# Autodesk Inventor assembly: microven
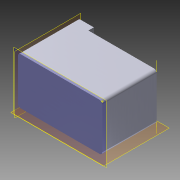
[picture p0: Inventor's stored thumbnail of the model, 180x180]
Saved by Autodesk Inventor 2015 (Build 190159000, 159)
## iProperties
Created: 2015-10-18
Part Number: microven
Document SubType Name: Assembly
Designer: omae
Author: omae
## Documents named in this file (2)
- C:\Users\omae\Desktop\研究室\論文・資料\ROS\kitchen\stl\microven.iam
- C:\Users\omae\Desktop\研究室\論文・資料\ROS\kitchen\toolinstall\homeIsland\summerSeminar\micorooven\microwaveOvenBox.ipt
## Components (1 placed, 1 different names)
1. microwaveOvenBox:1 — メイト:1, メイト:2, メイト:3
## Relationships (3: Mate 3)
- メイト:1 [Mate]: microwaveOvenBox:1
- メイト:2 [Mate]: microwaveOvenBox:1
- メイト:3 [Mate]: microwaveOvenBox:1
